# Autodesk Inventor assembly: złożenie gąsienicy lewej
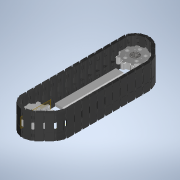
[picture p0: Inventor's stored thumbnail of the model, 180x180]
Saved by Autodesk Inventor 2021 (Build 250183000, 183)
## iProperties
Created: 2021-06-19
Part Number: złożenie gąsienicy lewej
Document SubType Name: Assembly
Designer: Łukasz
Author: Łukasz
## Documents named in this file (7)
- E:\GITHUB_Czołg\Szybki-Czolg-antyRadziecki\złożenie gąsienicy lewej.iam
- E:\GITHUB_Czołg\Szybki-Czolg-antyRadziecki\gąsienica.ipt
- E:\GITHUB_Czołg\Szybki-Czolg-antyRadziecki\koło napędowe.ipt
- E:\GITHUB_Czołg\Szybki-Czolg-antyRadziecki\koło łożyskowane.ipt
- E:\GITHUB_Czołg\Szybki-Czolg-antyRadziecki\dystans łożyska.ipt
- C:\Users\Łukasz\Documents\Inventor\Content Center Files\R2021\en-US\BS 292 (I)\BS 292 Part 1 - 6001 - 12 x 28 x 8.ipt
- E:\GITHUB_Czołg\Szybki-Czolg-antyRadziecki\mocowanie zawieszenia.ipt
## Components (43 placed, 6 different names)
1. gąsienica:1 — Rotational:1, Angle:1, Rotational:6, Angle:6
2. gąsienica:2 — Rotational:1, Angle:1, Rotational:2, Angle:2, Flush:4
3. gąsienica:3 — Rotational:5, Angle:5, Rotational:7, Angle:8
4. gąsienica:4 — Rotational:3, Angle:3, Rotational:4, Angle:4
5. gąsienica:5 — Rotational:2, Angle:2, Rotational:3, Angle:3, Mate:1, Flush:1
6. gąsienica:6 — Rotational:6, Angle:6, Rotational:9, Angle:7
7. gąsienica:7 — Rotational:4, Angle:4, Rotational:5, Angle:5
8. gąsienica:8 — Rotational:7, Rotational:8, Angle:8, Angle:9
9. gąsienica:9 — Rotational:8, Angle:9, Rotational:31, Angle:28
10. gąsienica:10 — Rotational:9, Angle:7, Rotational:10, Angle:10
11. koło napędowe:1 — Mate:1, Flush:1, Flush:3, Mate:2, Mate:3, Flush:4, Flush:5, Flush:6, Mate:4
12. koło łożyskowane:1 — Flush:3, Mate:2, Mate:3, Insert:1, Insert:2, Insert:3
13. dystans łożyska:1 — Insert:1
14. BS 292: Part 1 (I) (Metric) 6001 - 12 x 28 x 8:1 — Insert:2
15. BS 292: Part 1 (I) (Metric) 6001 - 12 x 28 x 8:2 — Insert:3
16. gąsienica:11 — Rotational:10, Rotational:11, Angle:10, Angle:11
17. gąsienica:12 — Rotational:11, Angle:11, Rotational:12, Angle:12
18. gąsienica:13 — Rotational:13, Rotational:14, Angle:13, Angle:14
19. gąsienica:14 — Rotational:14, Angle:14, Rotational:15, Angle:15
20. gąsienica:15 — Rotational:15, Rotational:16, Angle:15, Angle:16
21. gąsienica:16 — Rotational:12, Rotational:13, Angle:12, Angle:13
22. gąsienica:17 — Rotational:16, Angle:16, Rotational:17, Angle:17
23. gąsienica:18 — Rotational:17, Rotational:18, Angle:17, Angle:18
24. gąsienica:19 — Rotational:18, Angle:18, Rotational:19, Angle:19
25. gąsienica:20 — Rotational:19, Rotational:20, Angle:19, Angle:20
26. gąsienica:21 — Rotational:20, Angle:20, Rotational:21, Angle:21
27. gąsienica:22 — Rotational:21, Rotational:22, Angle:21, Angle:22
28. gąsienica:23 — Rotational:22, Angle:22, Rotational:23, Angle:23
29. gąsienica:24 — Rotational:23, Rotational:24, Angle:23, Angle:24
30. gąsienica:25 — Rotational:24, Angle:24, Rotational:25, Angle:25
31. gąsienica:26 — Rotational:25, Rotational:26, Angle:25, Angle:26
32. gąsienica:27 — Rotational:26, Rotational:27, Angle:26, Angle:27
33. gąsienica:28 — Rotational:27, Angle:27, Rotational:37, Angle:36
34. gąsienica:29 — Rotational:29, Angle:30, Rotational:32, Angle:32
35. gąsienica:30 — Rotational:29, Rotational:30, Angle:29, Angle:30
36. gąsienica:31 — Rotational:30, Rotational:31, Angle:28, Angle:29
37. gąsienica:32 — Rotational:32, Rotational:33, Angle:31, Angle:32
38. gąsienica:33 — Rotational:33, Angle:31, Rotational:34, Angle:33
39. gąsienica:34 — Rotational:34, Rotational:36, Angle:33, Angle:34
40. gąsienica:35 — Rotational:35, Angle:35, Rotational:38, Angle:37
41. gąsienica:36 — Rotational:35, Rotational:36, Angle:34, Angle:35
42. gąsienica:37 — Rotational:37, Angle:36, Rotational:38, Angle:37
43. mocowanie zawieszenia:1 — Flush:5, Flush:6, Mate:4
## Relationships (86: RevoluteJoint 37, Angle 37, Flush 5, Mate 4, Insert 3)
- Rotational:1 [RevoluteJoint]: gąsienica:1 ↔ gąsienica:2
- Angle:1 (-36 deg): gąsienica:1 ↔ gąsienica:2
- Rotational:2 [RevoluteJoint]: gąsienica:2 ↔ gąsienica:5
- Angle:2 (36 deg): gąsienica:2 ↔ gąsienica:5
- Rotational:3 [RevoluteJoint]: gąsienica:4 ↔ gąsienica:5
- Angle:3 (36 deg): gąsienica:4 ↔ gąsienica:5
- Rotational:4 [RevoluteJoint]: gąsienica:4 ↔ gąsienica:7
- Angle:4 (26 deg): gąsienica:4 ↔ gąsienica:7
- Rotational:5 [RevoluteJoint]: gąsienica:3 ↔ gąsienica:7
- Angle:5 (0 deg): gąsienica:3 ↔ gąsienica:7
- Rotational:6 [RevoluteJoint]: gąsienica:1 ↔ gąsienica:6
- Angle:6 (0 deg): gąsienica:1 ↔ gąsienica:6
- Rotational:7 [RevoluteJoint]: gąsienica:3 ↔ gąsienica:8
- Rotational:8 [RevoluteJoint]: gąsienica:8 ↔ gąsienica:9
- Rotational:9 [RevoluteJoint]: gąsienica:6 ↔ gąsienica:10
- Angle:7 (0 deg): gąsienica:6 ↔ gąsienica:10
- Angle:8 (22.893 deg): gąsienica:3 ↔ gąsienica:8
- Angle:9 (23.107 deg): gąsienica:8 ↔ gąsienica:9
- Mate:1 (1 mm): gąsienica:5 ↔ koło napędowe:1
- Flush:1: gąsienica:5 ↔ koło napędowe:1
- Flush:3: koło napędowe:1 ↔ koło łożyskowane:1
- Mate:2 (-325 mm): koło napędowe:1 ↔ koło łożyskowane:1
- Mate:3: koło napędowe:1 ↔ koło łożyskowane:1
- Insert:1 (8 mm): koło łożyskowane:1 ↔ dystans łożyska:1
- Insert:2: koło łożyskowane:1 ↔ BS 292: Part 1 (I) (Metric) 6001 - 12 x 28 x 8:1
- Insert:3: koło łożyskowane:1 ↔ BS 292: Part 1 (I) (Metric) 6001 - 12 x 28 x 8:2
- Rotational:10 [RevoluteJoint]: gąsienica:10 ↔ gąsienica:11
- Rotational:11 [RevoluteJoint]: gąsienica:11 ↔ gąsienica:12
- Angle:10 (0 deg): gąsienica:10 ↔ gąsienica:11
- Angle:11 (0 deg): gąsienica:11 ↔ gąsienica:12
- Rotational:12 [RevoluteJoint]: gąsienica:12 ↔ gąsienica:16
- Rotational:13 [RevoluteJoint]: gąsienica:13 ↔ gąsienica:16
- Rotational:14 [RevoluteJoint]: gąsienica:13 ↔ gąsienica:14
- Angle:12 (0 deg): gąsienica:12 ↔ gąsienica:16
- Angle:13 (0 deg): gąsienica:13 ↔ gąsienica:16
- Angle:14 (0 deg): gąsienica:13 ↔ gąsienica:14
- Rotational:15 [RevoluteJoint]: gąsienica:14 ↔ gąsienica:15
- Rotational:16 [RevoluteJoint]: gąsienica:15 ↔ gąsienica:17
- Angle:15 (0 deg): gąsienica:14 ↔ gąsienica:15
- Angle:16 (0 deg): gąsienica:15 ↔ gąsienica:17
- Rotational:17 [RevoluteJoint]: gąsienica:17 ↔ gąsienica:18
- Rotational:18 [RevoluteJoint]: gąsienica:18 ↔ gąsienica:19
- Angle:17 (0 deg): gąsienica:17 ↔ gąsienica:18
- Angle:18 (0 deg): gąsienica:18 ↔ gąsienica:19
- Rotational:19 [RevoluteJoint]: gąsienica:19 ↔ gąsienica:20
- Rotational:20 [RevoluteJoint]: gąsienica:20 ↔ gąsienica:21
- Angle:19 (0 deg): gąsienica:19 ↔ gąsienica:20
- Angle:20 (0 deg): gąsienica:20 ↔ gąsienica:21
- Rotational:21 [RevoluteJoint]: gąsienica:21 ↔ gąsienica:22
- Rotational:22 [RevoluteJoint]: gąsienica:22 ↔ gąsienica:23
- Angle:21 (36 deg): gąsienica:21 ↔ gąsienica:22
- Angle:22 (36 deg): gąsienica:22 ↔ gąsienica:23
- Rotational:23 [RevoluteJoint]: gąsienica:23 ↔ gąsienica:24
- Rotational:24 [RevoluteJoint]: gąsienica:24 ↔ gąsienica:25
- Angle:23 (36 deg): gąsienica:23 ↔ gąsienica:24
- Angle:24 (26 deg): gąsienica:24 ↔ gąsienica:25
- Rotational:25 [RevoluteJoint]: gąsienica:25 ↔ gąsienica:26
- Rotational:26 [RevoluteJoint]: gąsienica:26 ↔ gąsienica:27
- Rotational:27 [RevoluteJoint]: gąsienica:27 ↔ gąsienica:28
- Angle:25 (0 deg): gąsienica:25 ↔ gąsienica:26
- Angle:26 (22.893 deg): gąsienica:26 ↔ gąsienica:27
- Angle:27 (23.107 deg): gąsienica:27 ↔ gąsienica:28
- Rotational:29 [RevoluteJoint]: gąsienica:29 ↔ gąsienica:30
- Rotational:30 [RevoluteJoint]: gąsienica:30 ↔ gąsienica:31
- Rotational:31 [RevoluteJoint]: gąsienica:9 ↔ gąsienica:31
- Angle:28 (0 deg): gąsienica:9 ↔ gąsienica:31
- Angle:29 (0 deg): gąsienica:30 ↔ gąsienica:31
- Angle:30 (0 deg): gąsienica:29 ↔ gąsienica:30
- Rotational:32 [RevoluteJoint]: gąsienica:29 ↔ gąsienica:32
- Rotational:33 [RevoluteJoint]: gąsienica:32 ↔ gąsienica:33
- Angle:31 (0 deg): gąsienica:32 ↔ gąsienica:33
- Angle:32 (0 deg): gąsienica:29 ↔ gąsienica:32
- Rotational:34 [RevoluteJoint]: gąsienica:33 ↔ gąsienica:34
- Rotational:35 [RevoluteJoint]: gąsienica:35 ↔ gąsienica:36
- Rotational:36 [RevoluteJoint]: gąsienica:34 ↔ gąsienica:36
- Angle:33 (0 deg): gąsienica:33 ↔ gąsienica:34
- Angle:34 (0 deg): gąsienica:34 ↔ gąsienica:36
- Angle:35 (0 deg): gąsienica:35 ↔ gąsienica:36
- Rotational:37 [RevoluteJoint]: gąsienica:28 ↔ gąsienica:37
- Angle:36 (0 deg): gąsienica:28 ↔ gąsienica:37
- Rotational:38 [RevoluteJoint]: gąsienica:35 ↔ gąsienica:37
- Angle:37 (0 deg): gąsienica:35 ↔ gąsienica:37
- Flush:4: gąsienica:2 ↔ koło napędowe:1
- Flush:5 (6 mm): koło napędowe:1 ↔ mocowanie zawieszenia:1
- Flush:6 (62.5 mm): koło napędowe:1 ↔ mocowanie zawieszenia:1
- Mate:4: koło napędowe:1 ↔ mocowanie zawieszenia:1
